# Autodesk Inventor assembly: Hinge
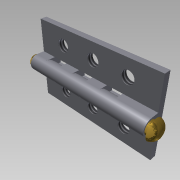
[picture p0: Inventor's stored thumbnail of the model, 180x180]
Saved by Autodesk Inventor 2012 (Build 160160000, 160)
## iProperties
Created: 2011-10-18
Part Number: Hinge
Document SubType Name: Assembly
Designer: Smeet
Author: Smeet
## Documents named in this file (4)
- C:\WORKSHOP\ADMETAL\sheet.metal.bin\predesign\Hinge\Hinge.iam
- C:\WORKSHOP\ADMETAL\sheet.metal.bin\predesign\Hinge\HingeP1.ipt
- C:\WORKSHOP\ADMETAL\sheet.metal.bin\predesign\Hinge\HingeP2.ipt
- C:\WORKSHOP\ADMETAL\sheet.metal.bin\predesign\Hinge\HingeBolt.ipt
## Components (3 placed, 3 different names)
1. HingeP1:1 — Mate:1, Mate:2, Insert:1, Angle:1
2. HingeP2:1 — Mate:1, Mate:2, Angle:1
3. HingeBolt:1 — Insert:1
## Relationships (4: Mate 2, Insert 1, Angle 1)
- Mate:1: HingeP1:1 ↔ HingeP2:1
- Mate:2: HingeP1:1 ↔ HingeP2:1
- Insert:1 (1.27 mm): HingeP1:1 ↔ HingeBolt:1
- Angle:1 (180 deg): HingeP1:1 ↔ HingeP2:1
